# Autodesk Inventor assembly: electronica carcasa
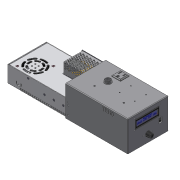
[picture p0: Inventor's stored thumbnail of the model, 180x180]
Saved by Autodesk Inventor 2019 (Build 230136000, 136)
## iProperties
Created: 2019-11-13
Part Number: electronica carcasa
Document SubType Name: Assembly
Designer: Carlos Andres garcia velez
Author: Carlos Andres garcia velez
## Documents named in this file (11)
- C:\Users\user\OneDrive\Carlos_2\02 TRABAJOS\MULTIPLO\Conveyor\ELECTRONICA\electronica carcasa.iam
- C:\Users\user\OneDrive\Carlos_2\02 TRABAJOS\MULTIPLO\Conveyor\ELECTRONICA\LCD.iam
- C:\Users\user\OneDrive\Carlos_2\02 TRABAJOS\MULTIPLO\Conveyor\ELECTRONICA\SMAKN TB6600 STEPPER MOTOR DRIVER.iam
- C:\Users\user\OneDrive\Carlos_2\02 TRABAJOS\MULTIPLO\Conveyor\ELECTRONICA\SCHEDA RELE' 2 CANALI.iam
- C:\Users\user\OneDrive\Carlos_2\02 TRABAJOS\MULTIPLO\Conveyor\ELECTRONICA\Pulse_power_supply_36V_600W.iam
- C:\Users\user\OneDrive\Carlos_2\02 TRABAJOS\MULTIPLO\Conveyor\ELECTRONICA\Power Supply S-60-12 v2.iam
- C:\Users\user\OneDrive\Carlos_2\02 TRABAJOS\MULTIPLO\Conveyor\ELECTRONICA\arduino-nano-shield-cnc-1.snapshot.4 (1)\nano shield.iam
- C:\Users\user\OneDrive\Carlos_2\02 TRABAJOS\MULTIPLO\Conveyor\ELECTRONICA\Rotary Encoder EC11\ROTARY_ENCODER_EC11.iam
- C:\Users\user\OneDrive\Carlos_2\02 TRABAJOS\MULTIPLO\Conveyor\ELECTRONICA\carcasa.ipt
- C:\Users\user\OneDrive\Carlos_2\02 TRABAJOS\MULTIPLO\Conveyor\ELECTRONICA\AC Receptacle NEMA 5-15 - PN SS-6B.ipt
- C:\Users\user\OneDrive\Carlos_2\02 TRABAJOS\MULTIPLO\Conveyor\ELECTRONICA\ficha audio panel 4p.ipt
## Components (10 placed, 10 different names)
1. LCD:1 [sub-assembly] — Mate:15, Mate:16, Mate:29
2. SMAKN TB6600 STEPPER MOTOR DRIVER:1 [sub-assembly] — Mate:12, Mate:13, Mate:14
3. SCHEDA RELE' 2 CANALI:1 [sub-assembly] — Mate:21, Mate:22, Mate:23
4. Pulse_power_supply_36V_600W:1 [sub-assembly] — Flush:1, Mate:1, Mate:10, Mate:11, Mate:13
5. Power Supply S-60-12 v2:1 [sub-assembly] — Flush:1, Mate:1, Mate:9
6. nano shield:1 [sub-assembly] — Mate:19, Flush:2, Mate:20
7. ROTARY_ENCODER_EC11:1 [sub-assembly] — Mate:17, Mate:24, Flush:3
8. carcasa:1 — Mate:9, Mate:10, Mate:11, Mate:12, Mate:14, Mate:15, Mate:16, Mate:17, Mate:19, Flush:2, Mate:20, Mate:21, Mate:22, Mate:23, Mate:24, Flush:3, Mate:25, Flush:4, Flush:5, Mate:26, Mate:27, Mate:28, Mate:29
9. AC Receptacle NEMA 5-15 - PN SS-6B:1 — Mate:25, Flush:4, Flush:5
10. ficha audio panel 4p:1 — Mate:26, Mate:27, Mate:28
## Relationships (26: Mate 21, Flush 5)
- Flush:1: Pulse_power_supply_36V_600W:1 ↔ Power Supply S-60-12 v2:1
- Mate:1: Pulse_power_supply_36V_600W:1 ↔ Power Supply S-60-12 v2:1
- Mate:9 (4 mm): Power Supply S-60-12 v2:1 ↔ carcasa:1
- Mate:10: Pulse_power_supply_36V_600W:1 ↔ carcasa:1
- Mate:11: Pulse_power_supply_36V_600W:1 ↔ carcasa:1
- Mate:12: SMAKN TB6600 STEPPER MOTOR DRIVER:1 ↔ carcasa:1
- Mate:13 (15 mm): SMAKN TB6600 STEPPER MOTOR DRIVER:1 ↔ Pulse_power_supply_36V_600W:1
- Mate:14 (10 mm): SMAKN TB6600 STEPPER MOTOR DRIVER:1 ↔ carcasa:1
- Mate:15 (5 mm): LCD:1 ↔ carcasa:1
- Mate:16 (3 mm): LCD:1 ↔ carcasa:1
- Mate:17 (5 mm): ROTARY_ENCODER_EC11:1 ↔ carcasa:1
- Mate:19 (3.2 mm): nano shield:1 ↔ carcasa:1
- Flush:2 (3 mm): nano shield:1 ↔ carcasa:1
- Mate:20 (1 mm): nano shield:1 ↔ carcasa:1
- Mate:21 (3 mm): SCHEDA RELE' 2 CANALI:1 ↔ carcasa:1
- Mate:22 (25 mm): SCHEDA RELE' 2 CANALI:1 ↔ carcasa:1
- Mate:23 (30 mm): SCHEDA RELE' 2 CANALI:1 ↔ carcasa:1
- Mate:24 (50 mm): ROTARY_ENCODER_EC11:1 ↔ carcasa:1
- Flush:3 (10 mm): ROTARY_ENCODER_EC11:1 ↔ carcasa:1
- Mate:25: carcasa:1 ↔ AC Receptacle NEMA 5-15 - PN SS-6B:1
- Flush:4 (8 mm): carcasa:1 ↔ AC Receptacle NEMA 5-15 - PN SS-6B:1
- Flush:5 (50 mm): carcasa:1 ↔ AC Receptacle NEMA 5-15 - PN SS-6B:1
- Mate:26: carcasa:1 ↔ ficha audio panel 4p:1
- Mate:27 (-55 mm): carcasa:1 ↔ ficha audio panel 4p:1
- Mate:28 (-60 mm): carcasa:1 ↔ ficha audio panel 4p:1
- Mate:29 (15 mm): LCD:1 ↔ carcasa:1
